# Autodesk Inventor assembly: HbIndexFinger01ForChild_MIR1
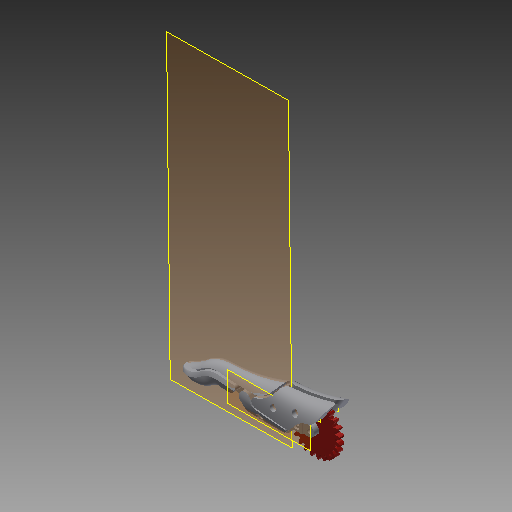
[picture p0: Inventor's stored thumbnail of the model, 512x512]
Saved by Autodesk Inventor 2017.3 (Build 213256000, 256)
## iProperties
Part Number: HbIndexFinger01ForChild_MIR1
Material: 一般
Document SubType Name: Assembly
Designer: sktom
Author: sktom
## Documents named in this file (10)
- D:\CloudStrage\OneDrive\CAD\MAJ\hackberry\HACKberry-hardware\3D_69%inlength\Inventor\HbHandForChild\HbIndexFinger01ForChild\HbIndexFinger01ForChild_MIR1.iam
- D:\CloudStrage\OneDrive\CAD\MAJ\hackberry\HACKberry-hardware\3D_69%inlength\Inventor\HbHandForChild\HbIndexFinger01ForChild\HbIndexInputLink02ForChild_MIR1.ipt
- D:\CloudStrage\OneDrive\CAD\MAJ\hackberry\HACKberry-hardware\3D_69%inlength\Inventor\HbHandForChild\HbIndexFinger01ForChild\HbIndexMiddle-DistalPhalanx02ForChild_MIR1.ipt
- D:\CloudStrage\OneDrive\CAD\MAJ\hackberry\HACKberry-hardware\3D_69%inlength\Inventor\HbHandForChild\HbIndexFinger01ForChild\HbIndexCouplerLink02ForChild_MIR1.ipt
- D:\CloudStrage\OneDrive\CAD\MAJ\hackberry\HACKberry-hardware\3D_69%inlength\Inventor\HbHandForChild\HbIndexFinger01ForChild\HbIndexCouplerLinkCover02ForChild_MIR1.ipt
- D:\CloudStrage\OneDrive\CAD\MAJ\hackberry\HACKberry-hardware\3D_69%inlength\Inventor\HbHandForChild\HbIndexFinger01ForChild\HbIndexProximalPhalanx03ForChild_MIR1.ipt
- D:\CloudStrage\OneDrive\CAD\MAJ\hackberry\HACKberry-hardware\3D_69%inlength\Inventor\HbHandForChild\HbIndexFinger01ForChild\HbIndexProximalPhalanxCover02ForChild_MIR1.ipt
- D:\CloudStrage\OneDrive\CAD\MAJ\hackberry\HACKberry-hardware\3D_69%inlength\Inventor\HbHandForChild\HbIndexFinger01ForChild\HbIndexReleaseLever02ForChild_MIR1.ipt
- D:\CloudStrage\OneDrive\CAD\MAJ\hackberry\HACKberry-hardware\3D_69%inlength\Inventor\HbHandForChild\HbIndexFinger01ForChild\Spur Gear (24 teeth)_MIR.ipt
- D:\CloudStrage\OneDrive\CAD\MAJ\hackberry\HACKberry-hardware\3D_69%inlength\Inventor\HbHandForChild\HbIndexFinger01ForChild\shaft_phi1.5_l6_MIR.ipt
## Components (12 placed, 9 different names)
1. HbIndexInputLink02ForChild_MIR1:1 — 挿入:4, 円柱状:3, 円柱状:1
2. HbIndexMiddle-DistalPhalanx02ForChild_MIR1:1 — 挿入:1, 挿入:5, 円柱状:2
3. HbIndexCouplerLink02ForChild_MIR1:1 — 挿入:4, 挿入:1, 挿入:3, 挿入:2, 挿入:12, 挿入:14
4. HbIndexCouplerLinkCover02ForChild_MIR1:1 — 挿入:3, 挿入:2, 挿入:10
5. HbIndexProximalPhalanx03ForChild_MIR1:1 — 挿入:9, 円柱状:3, 円柱状:2
6. HbIndexProximalPhalanxCover02ForChild_MIR1:1 — 挿入:5, 挿入:8, 挿入:11, 挿入:13, 円柱状:1
7. HbIndexReleaseLever02ForChild_MIR1:1 — 挿入:8
8. Spur Gear (24 teeth)_MIR:1 — 挿入:10, 挿入:9
9. shaft_phi1.5_l6_MIR:1 — 挿入:11
10. shaft_phi1.5_l6_MIR:2 — 挿入:12
11. shaft_phi1.5_l6_MIR:3 — 挿入:13
12. shaft_phi1.5_l6_MIR:4 — 挿入:14
## Relationships (15: Insert 12, CylindricalJoint 3)
- 挿入:4 [Insert] (0.25 mm): HbIndexInputLink02ForChild_MIR1:1 ↔ HbIndexCouplerLink02ForChild_MIR1:1
- 挿入:1 [Insert] (0.4 mm): HbIndexMiddle-DistalPhalanx02ForChild_MIR1:1 ↔ HbIndexCouplerLink02ForChild_MIR1:1
- 挿入:3 [Insert]: HbIndexCouplerLink02ForChild_MIR1:1 ↔ HbIndexCouplerLinkCover02ForChild_MIR1:1
- 挿入:2 [Insert]: HbIndexCouplerLink02ForChild_MIR1:1 ↔ HbIndexCouplerLinkCover02ForChild_MIR1:1
- 挿入:5 [Insert] (0.4 mm): HbIndexMiddle-DistalPhalanx02ForChild_MIR1:1 ↔ HbIndexProximalPhalanxCover02ForChild_MIR1:1
- 挿入:8 [Insert] (0.2 mm): HbIndexProximalPhalanxCover02ForChild_MIR1:1 ↔ HbIndexReleaseLever02ForChild_MIR1:1
- 挿入:10 [Insert]: HbIndexCouplerLinkCover02ForChild_MIR1:1 ↔ Spur Gear (24 teeth)_MIR:1
- 挿入:9 [Insert]: HbIndexProximalPhalanx03ForChild_MIR1:1 ↔ Spur Gear (24 teeth)_MIR:1
- 挿入:11 [Insert] (0.5 mm): HbIndexProximalPhalanxCover02ForChild_MIR1:1 ↔ shaft_phi1.5_l6_MIR:1
- 挿入:12 [Insert] (0.5 mm): HbIndexCouplerLink02ForChild_MIR1:1 ↔ shaft_phi1.5_l6_MIR:2
- 挿入:13 [Insert] (0.5 mm): HbIndexProximalPhalanxCover02ForChild_MIR1:1 ↔ shaft_phi1.5_l6_MIR:3
- 挿入:14 [Insert] (-2 mm): HbIndexCouplerLink02ForChild_MIR1:1 ↔ shaft_phi1.5_l6_MIR:4
- 円柱状:3 [CylindricalJoint]: HbIndexInputLink02ForChild_MIR1:1 ↔ HbIndexProximalPhalanx03ForChild_MIR1:1
- 円柱状:2 [CylindricalJoint]: HbIndexMiddle-DistalPhalanx02ForChild_MIR1:1 ↔ HbIndexProximalPhalanx03ForChild_MIR1:1
- 円柱状:1 [CylindricalJoint]: HbIndexInputLink02ForChild_MIR1:1 ↔ HbIndexProximalPhalanxCover02ForChild_MIR1:1
